# Autodesk Inventor assembly: joint_hip_MIR
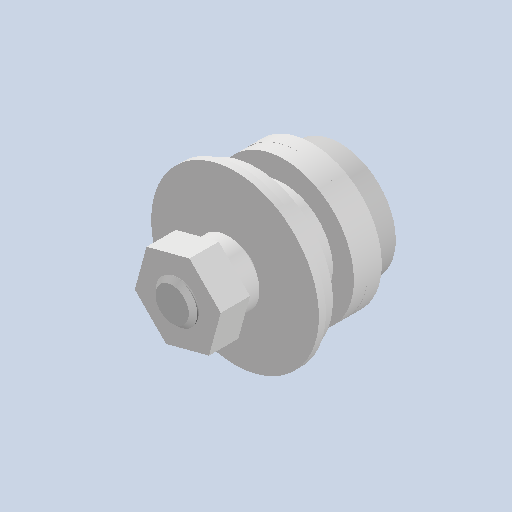
[picture p0: Inventor's stored thumbnail of the model, 512x512]
Saved by Autodesk Inventor 2022 (Build 260153000, 153)
## iProperties
Created: 2022-10-13
Part Number: joint_hip_MIR
Document SubType Name: Assembly
Designer: haya
Author: haya
## Documents named in this file (7)
- C:\Users\haya\Documents\GitHub\OpenPlatform_ver3_0 - コピー\joint_hip_MIR.iam
- C:\Users\haya\Documents\GitHub\OpenPlatform_ver3_0 - コピー\S3-15-3W_MIR.ipt
- C:\Users\haya\Documents\GitHub\OpenPlatform_ver3_0 - コピー\80F-0503_MIR.ipt
- C:\Users\haya\Documents\GitHub\OpenPlatform_ver3_0 - コピー\AAW-0510-10_MIR.ipt
- C:\Users\haya\Documents\GitHub\OpenPlatform_ver3_0 - コピー\LL-7211-10_MIR.ipt
- C:\Users\haya\Documents\GitHub\OpenPlatform_ver3_0 - コピー\DBB3-5-5_MIR.ipt
- C:\Users\haya\Documents\GitHub\OpenPlatform_ver3_0 - コピー\UUW-0312-5H_MIR.ipt
## Components (6 placed, 6 different names)
1. S3-15-3W_MIR:1 — 挿入:4
2. 80F-0503_MIR:1 — 挿入:1, 挿入:2, 挿入:3
3. AAW-0510-10_MIR:1 — 挿入:1, 挿入:5
4. LL-7211-10_MIR:1 — 挿入:2
5. DBB3-5-5_MIR:1 — 挿入:5
6. UUW-0312-5H_MIR:1 — 挿入:3, 挿入:4
## Relationships (5: Insert 5)
- 挿入:1 [Insert]: 80F-0503_MIR:1 ↔ AAW-0510-10_MIR:1
- 挿入:2 [Insert]: 80F-0503_MIR:1 ↔ LL-7211-10_MIR:1
- 挿入:5 [Insert]: AAW-0510-10_MIR:1 ↔ DBB3-5-5_MIR:1
- 挿入:3 [Insert]: 80F-0503_MIR:1 ↔ UUW-0312-5H_MIR:1
- 挿入:4 [Insert] (2 mm): S3-15-3W_MIR:1 ↔ UUW-0312-5H_MIR:1
